# Autodesk Inventor assembly: Assembly1
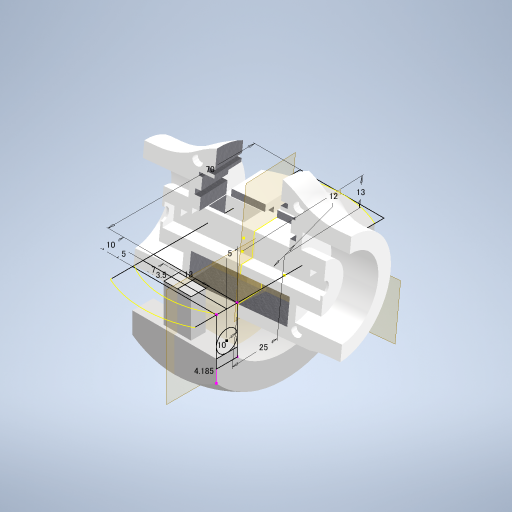
[picture p0: Inventor's stored thumbnail of the model, 512x512]
Saved by Autodesk Inventor 2023 (Build 270158000, 158)
## iProperties
Created: 2022-12-16
Part Number: Assembly1
Document SubType Name: Assembly
Designer: ellie
Author: ellie
## Documents named in this file (3)
- C:\Users\ellie\Documents\github\tanekonsat2022_runback\machinary\parts\tale\Assembly1.iam
- C:\Users\ellie\Documents\github\tanekonsat2022_runback\machinary\parts\tale\tail12.16.ipt
- C:\Users\ellie\Documents\github\tanekonsat2022_runback\machinary\body\body back\back moter middle tire ver\back moter lemon tale.ipt
## Components (2 placed, 2 different names)
1. tail12.16:1 — メイト:1
2. body moter middle:1 — メイト:1
## Relationships (1: Mate 1)
- メイト:1 [Mate]: tail12.16:1 ↔ body moter middle:1
